# Autodesk Inventor assembly: base.assembly
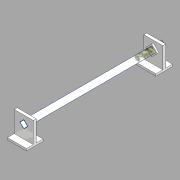
[picture p0: Inventor's stored thumbnail of the model, 180x180]
Saved by Autodesk Inventor 2020 (Build 240168000, 168)
## iProperties
Created: 2021-04-02
Part Number: base.assembly
Document SubType Name: Assembly
Designer: griss
Author: griss
## Documents named in this file (3)
- C:\Users\griss\Documents\Inventor\CNC\y_axis_base\base.assembly.iam
- C:\Users\griss\Documents\Inventor\CNC\y_axis_base\base_rail.ipt
- C:\Users\griss\Documents\Inventor\CNC\y_axis_base\base_end_mounts.ipt
## Components (3 placed, 2 different names)
1. base_rail:1 — Flush:1, Mate:1, Mate:2, Flush:2, Mate:3, Mate:4
2. base_end_mounts:1 — Flush:1, Mate:1, Mate:2
3. base_end_mounts:2 — Flush:2, Mate:3, Mate:4
## Relationships (6: Mate 4, Flush 2)
- Flush:1 (25.4 mm): base_rail:1 ↔ base_end_mounts:1
- Mate:1: base_rail:1 ↔ base_end_mounts:1
- Mate:2: base_rail:1 ↔ base_end_mounts:1
- Flush:2: base_rail:1 ↔ base_end_mounts:2
- Mate:3: base_rail:1 ↔ base_end_mounts:2
- Mate:4: base_rail:1 ↔ base_end_mounts:2
